# Autodesk Inventor assembly: NMR Frame
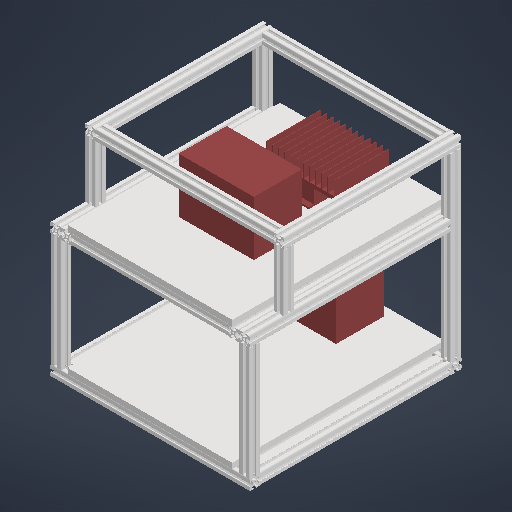
[picture p0: Inventor's stored thumbnail of the model, 512x512]
Saved by Autodesk Inventor 2026.2 (Build 302298010, 298A)
## iProperties
Created: 2026-08-09
Part Number: NMR Frame
Document SubType Name: Assembly
Designer: aiden
Author: aiden
## Documents named in this file (14)
- D:\[GitHub]\flowthrough-water-quality-monitoring-system\system_development\Moultrie\v0.4.1\NMRtray 8_24_2026\Frame\NMR Frame.iam
- D:\[GitHub]\flowthrough-water-quality-monitoring-system\system_development\Moultrie\v0.4.1\NMRtray 8_24_2026\Al Bars\AL369.575_5537T104.ipt
- D:\[GitHub]\flowthrough-water-quality-monitoring-system\system_development\Moultrie\v0.4.1\NMRtray 8_24_2026\Al Bars\AL210_5537T104.ipt
- D:\[GitHub]\flowthrough-water-quality-monitoring-system\system_development\Moultrie\v0.4.1\NMRtray 8_24_2026\Al Bars\AL336_5537T104.ipt
- D:\[GitHub]\flowthrough-water-quality-monitoring-system\system_development\Moultrie\v0.4.1\NMRtray 8_24_2026\Al Bars\AL329.575_5537T104.ipt
- D:\[GitHub]\flowthrough-water-quality-monitoring-system\system_development\Moultrie\v0.4.1\NMRtray 8_24_2026\Al Bars\AL106_5537T104.ipt
- D:\[GitHub]\flowthrough-water-quality-monitoring-system\system_development\Moultrie\v0.4.1\NMRtray 8_24_2026\Al Bars\AL373.7_5537T104.ipt
- D:\[GitHub]\flowthrough-water-quality-monitoring-system\system_development\Moultrie\v0.4.1\NMRtray 8_24_2026\Al Bars\AL393.7_5537T104.ipt
- D:\[GitHub]\flowthrough-water-quality-monitoring-system\system_development\Moultrie\v0.4.1\NMRtray 8_24_2026\Al Bars\AL289.575_5537T104.ipt
- D:\[GitHub]\flowthrough-water-quality-monitoring-system\system_development\Moultrie\v0.4.1\NMRtray 8_24_2026\Al Bars\20x40_353.7.ipt
- D:\[GitHub]\flowthrough-water-quality-monitoring-system\system_development\Moultrie\v0.4.1\NMRtray 8_24_2026\Shelf.ipt
- D:\[GitHub]\flowthrough-water-quality-monitoring-system\system_development\Moultrie\v0.4.1\NMRtray 8_24_2026\Electrical Components\Magnet.ipt
- D:\[GitHub]\flowthrough-water-quality-monitoring-system\system_development\Moultrie\v0.4.1\NMRtray 8_24_2026\Electrical Components\Heatsink and Amplifier.ipt
- D:\[GitHub]\flowthrough-water-quality-monitoring-system\system_development\Moultrie\v0.4.1\NMRtray 8_24_2026\Electrical Components\NMR Control Circuit Board.ipt
## Components (28 placed, 13 different names)
1. AL369.575_5537T104:1 — Rigid:4, Rigid:5, Mate:31, Flush:19, Mate:32, Flush:22, Mate:34, Flush:32, Mate:41
2. AL369.575_5537T104:2 — Rigid:6, Rigid:7, Mate:36
3. AL210_5537T104:1 — Rigid:5, Mate:21, Flush:8, Flush:21, Flush:26, Mate:42
4. AL210_5537T104:2 — Rigid:4, Mate:19, Flush:7, Flush:20, Flush:25
5. AL336_5537T104:1 — Rigid:6, Mate:10, Angle:3, Mate:18, Angle:6
6. AL336_5537T104:2 — Rigid:7, Mate:8, Angle:2, Mate:20
7. AL106_5537T104:1 — Mate:8, Mate:12, Angle:1, Flush:3, Mate:30, Flush:18, Mate:40
8. AL106_5537T104:2 — Mate:10, Mate:13, Flush:4, Mate:29, Flush:17
9. AL329.575_5537T104:2 — Mate:12, Angle:1, Flush:3, Angle:2
10. AL329.575_5537T104:3 — Mate:13, Flush:4, Angle:3, Mate:14, Angle:4, Flush:5, Mate:15, Flush:6, Angle:5
11. AL329.575_5537T104:4 — Mate:14, Angle:4, Flush:5
12. AL329.575_5537T104:5 — Mate:15, Flush:6, Angle:5
13. AL373.7_5537T104:1 — Mate:20, Mate:21, Flush:8, Mate:22, Flush:9, Flush:10, Mate:30, Flush:18, Flush:26, Mate:39
14. AL373.7_5537T104:2 — Mate:18, Mate:19, Flush:7, Mate:23, Flush:11, Flush:12, Mate:29, Flush:17, Flush:25
15. AL393.7_5537T104:1 — Mate:23, Flush:11, Flush:12
16. AL393.7_5537T104:2 — Mate:22, Flush:9, Flush:10, Mate:24, Flush:13, Flush:14, Mate:37, Flush:27, Flush:28, Mate:38, Flush:29, Flush:30
17. AL289.575_5537T104:1 — Mate:24, Flush:13, Flush:14
18. 20x40_353.7:1 — Mate:31, Flush:19, Flush:20, Mate:33, Flush:23, Mate:35, Flush:24
19. 20x40_353.7:2 — Mate:32, Flush:21, Flush:22
20. AL289.575_5537T104:2 — Mate:33, Flush:23, Mate:34
21. AL289.575_5537T104:3 — Mate:35, Flush:24, Mate:36
22. AL289.575_5537T104:4 — Mate:37, Flush:27, Flush:28, Flush:31
23. AL289.575_5537T104:5 — Mate:38, Flush:29, Flush:30
24. Shelf:1 — Flush:31, Mate:39, Mate:40, Mate:43, Mate:44
25. Shelf:2 — Flush:32, Mate:41, Mate:42, Mate:45
26. Magnet:1 — Mate:45, Angle:6
27. Heatsink and Amplifier:1 — Mate:43
28. NMR Control Circuit Board:1 — Mate:44
## Relationships (68: Mate 30, Flush 28, Angle 6, WeldJoint 4)
- Rigid:4 [WeldJoint]: AL369.575_5537T104:1 ↔ AL210_5537T104:2
- Rigid:5 [WeldJoint]: AL369.575_5537T104:1 ↔ AL210_5537T104:1
- Rigid:6 [WeldJoint]: AL369.575_5537T104:2 ↔ AL336_5537T104:1
- Rigid:7 [WeldJoint]: AL369.575_5537T104:2 ↔ AL336_5537T104:2
- Mate:8 (290 mm): AL336_5537T104:2 ↔ AL106_5537T104:1
- Mate:10 (290 mm): AL336_5537T104:1 ↔ AL106_5537T104:2
- Mate:12: AL106_5537T104:1 ↔ AL329.575_5537T104:2
- Angle:1 (0 deg): AL106_5537T104:1 ↔ AL329.575_5537T104:2
- Flush:3: AL106_5537T104:1 ↔ AL329.575_5537T104:2
- Angle:2 (0 deg): AL336_5537T104:2 ↔ AL329.575_5537T104:2
- Mate:13: AL106_5537T104:2 ↔ AL329.575_5537T104:3
- Flush:4: AL106_5537T104:2 ↔ AL329.575_5537T104:3
- Angle:3 (0 deg): AL336_5537T104:1 ↔ AL329.575_5537T104:3
- Mate:14: AL329.575_5537T104:3 ↔ AL329.575_5537T104:4
- Angle:4 (90 deg): AL329.575_5537T104:3 ↔ AL329.575_5537T104:4
- Flush:5: AL329.575_5537T104:3 ↔ AL329.575_5537T104:4
- Mate:15: AL329.575_5537T104:3 ↔ AL329.575_5537T104:5
- Flush:6: AL329.575_5537T104:3 ↔ AL329.575_5537T104:5
- Angle:5 (90 deg): AL329.575_5537T104:3 ↔ AL329.575_5537T104:5
- Mate:18: AL336_5537T104:1 ↔ AL373.7_5537T104:2
- Mate:19: AL210_5537T104:2 ↔ AL373.7_5537T104:2
- Flush:7: AL210_5537T104:2 ↔ AL373.7_5537T104:2
- Mate:20: AL336_5537T104:2 ↔ AL373.7_5537T104:1
- Mate:21: AL210_5537T104:1 ↔ AL373.7_5537T104:1
- Flush:8: AL210_5537T104:1 ↔ AL373.7_5537T104:1
- Mate:22: AL373.7_5537T104:1 ↔ AL393.7_5537T104:2
- Flush:9: AL373.7_5537T104:1 ↔ AL393.7_5537T104:2
- Flush:10: AL373.7_5537T104:1 ↔ AL393.7_5537T104:2
- Mate:23: AL373.7_5537T104:2 ↔ AL393.7_5537T104:1
- Flush:11: AL373.7_5537T104:2 ↔ AL393.7_5537T104:1
- Flush:12: AL373.7_5537T104:2 ↔ AL393.7_5537T104:1
- Mate:24 (10 mm): AL393.7_5537T104:2 ↔ AL289.575_5537T104:1
- Flush:13: AL393.7_5537T104:2 ↔ AL289.575_5537T104:1
- Flush:14 (-196.85 mm): AL393.7_5537T104:2 ↔ AL289.575_5537T104:1
- Mate:29: AL106_5537T104:2 ↔ AL373.7_5537T104:2
- Flush:17: AL106_5537T104:2 ↔ AL373.7_5537T104:2
- Mate:30: AL106_5537T104:1 ↔ AL373.7_5537T104:1
- Flush:18: AL106_5537T104:1 ↔ AL373.7_5537T104:1
- Mate:31: AL369.575_5537T104:1 ↔ 20x40_353.7:1
- Flush:19: AL369.575_5537T104:1 ↔ 20x40_353.7:1
- Flush:20: AL210_5537T104:2 ↔ 20x40_353.7:1
- Mate:32: AL369.575_5537T104:1 ↔ 20x40_353.7:2
- Flush:21: AL210_5537T104:1 ↔ 20x40_353.7:2
- Flush:22: AL369.575_5537T104:1 ↔ 20x40_353.7:2
- Mate:33: 20x40_353.7:1 ↔ AL289.575_5537T104:2
- Flush:23: 20x40_353.7:1 ↔ AL289.575_5537T104:2
- Mate:34 (88.425 mm): AL369.575_5537T104:1 ↔ AL289.575_5537T104:2
- Mate:35: 20x40_353.7:1 ↔ AL289.575_5537T104:3
- Flush:24: 20x40_353.7:1 ↔ AL289.575_5537T104:3
- Flush:25: AL210_5537T104:2 ↔ AL373.7_5537T104:2
- Flush:26: AL210_5537T104:1 ↔ AL373.7_5537T104:1
- Mate:36 (88.425 mm): AL369.575_5537T104:2 ↔ AL289.575_5537T104:3
- Mate:37: AL393.7_5537T104:2 ↔ AL289.575_5537T104:4
- Flush:27: AL393.7_5537T104:2 ↔ AL289.575_5537T104:4
- Flush:28: AL393.7_5537T104:2 ↔ AL289.575_5537T104:4
- Mate:38: AL393.7_5537T104:2 ↔ AL289.575_5537T104:5
- Flush:29: AL393.7_5537T104:2 ↔ AL289.575_5537T104:5
- Flush:30: AL393.7_5537T104:2 ↔ AL289.575_5537T104:5
- Flush:31: AL289.575_5537T104:4 ↔ Shelf:1
- Mate:39: AL373.7_5537T104:1 ↔ Shelf:1
- Mate:40 (12.5 mm): AL106_5537T104:1 ↔ Shelf:1
- Flush:32: AL369.575_5537T104:1 ↔ Shelf:2
- Mate:41: AL369.575_5537T104:1 ↔ Shelf:2
- Mate:42 (12.5 mm): AL210_5537T104:1 ↔ Shelf:2
- Mate:43: Shelf:1 ↔ Heatsink and Amplifier:1
- Mate:44: Shelf:1 ↔ NMR Control Circuit Board:1
- Mate:45: Shelf:2 ↔ Magnet:1
- Angle:6 (0 deg): AL336_5537T104:1 ↔ Magnet:1
